# Autodesk Inventor assembly: 圆筒储弹仓装配
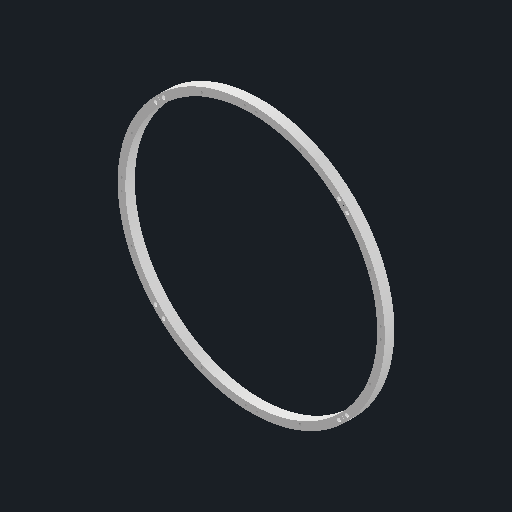
[picture p0: Inventor's stored thumbnail of the model, 512x512]
Saved by Autodesk Inventor 2025 (Build 290162000, 162)
## iProperties
Created: 2025-02-22
Part Number: 圆筒储弹仓装配
Document SubType Name: Assembly
Designer: XH
Author: XH
## Documents named in this file (2)
- C:\1A_Engineering_files\GCG全向轮步兵\云台\圆筒储弹仓装配.iam
- C:\1A_Engineering_files\GCG全向轮步兵\云台\组合.ipt
## Components (4 placed, 1 different names)
1. 组合:1 — 配合:1, 表面齐平:1
2. 组合:2 — 配合:1, 表面齐平:1, 配合:2, 表面齐平:2
3. 组合:3 — 配合:2, 表面齐平:2, 配合:3, 表面齐平:3
4. 组合:4 — 配合:3, 表面齐平:3
## Relationships (6: Mate 3, Flush 3)
- 配合:1 [Mate]: 组合:1 ↔ 组合:2
- 表面齐平:1 [Flush]: 组合:1 ↔ 组合:2
- 配合:2 [Mate]: 组合:2 ↔ 组合:3
- 表面齐平:2 [Flush]: 组合:2 ↔ 组合:3
- 配合:3 [Mate]: 组合:3 ↔ 组合:4
- 表面齐平:3 [Flush]: 组合:3 ↔ 组合:4
